# Autodesk Inventor assembly: 39079
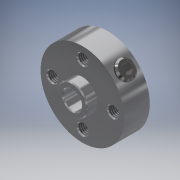
[picture p0: Inventor's stored thumbnail of the model, 180x180]
Saved by Autodesk Inventor 2019 (Build 230136000, 136)
## iProperties
Category: Wheel Hardware
Company: Autodesk Inc.
Created: 2017-01-02
Part Number: 39079
Document SubType Name: Assembly
Designer: Autodesk Inc.
Catalog Web Link: http://www.tetrixrobotics.com/TETRIX_Motor_Shaft_Hubs
Vendor: Tetrix
Author: Autodesk Inc.
## Documents named in this file (3)
- C:\Users\tbloo\Documents\Inventor\FTC Tetrix KOP\Tetrix_39079.iam
- C:\Users\tbloo\Downloads\FTC Tetrix KOP\Miscellaneous\Tetrix_39172_Collar.ipt
- C:\Users\tbloo\Downloads\FTC Tetrix KOP\Miscellaneous\Tetrix_39079_Screw.ipt
## Components (2 placed, 2 different names)
1. Tetrix_39079_Collar:1 — Mate:1
2. Tetrix_39079_Screw:1 — Mate:1
## Relationships (1: Mate 1)
- Mate:1: Tetrix_39079_Collar:1 ↔ Tetrix_39079_Screw:1
